# Autodesk Inventor assembly: Sneak100_Zeta
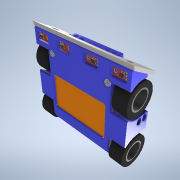
[picture p0: Inventor's stored thumbnail of the model, 180x180]
Saved by Autodesk Inventor 2021 (Build 250183000, 183)
## iProperties
Created: 2021-05-13
Part Number: Sneak100_Zeta
Document SubType Name: Assembly
Designer: ermoz
Author: ermoz
## Documents named in this file (15)
- D:\Moje Wyczyny\My_Poor_Projects\Sneak100_MiniSumo\minisumo-sneak100\mechanics\Sneak100_Zeta.iam
- D:\Moje Wyczyny\My_Poor_Projects\Sneak100_MiniSumo\minisumo-sneak100\mechanics\PreMadeParts\Pololu_MotorEncoderModule.iam
- D:\Moje Wyczyny\My_Poor_Projects\Sneak100_MiniSumo\minisumo-sneak100\mechanics\PreMadeParts\LiPO_2S_58x32x10.ipt
- D:\Moje Wyczyny\My_Poor_Projects\Sneak100_MiniSumo\minisumo-sneak100\mechanics\PreMadeParts\Solarbotics_RW2i.ipt
- D:\Moje Wyczyny\My_Poor_Projects\Sneak100_MiniSumo\minisumo-sneak100\mechanics\MechanicalElements\HullBottom.ipt
- D:\Moje Wyczyny\My_Poor_Projects\Sneak100_MiniSumo\minisumo-sneak100\mechanics\MechanicalElements\BatteryPlate.ipt
- D:\Moje Wyczyny\My_Poor_Projects\Sneak100_MiniSumo\minisumo-sneak100\mechanics\PreMadeParts\QTR1A.iam
- D:\Moje Wyczyny\My_Poor_Projects\Sneak100_MiniSumo\minisumo-sneak100\mechanics\PreMadeParts\M3_Short_Bolt.ipt
- D:\Moje Wyczyny\My_Poor_Projects\Sneak100_MiniSumo\minisumo-sneak100\mechanics\ModyfiedParts\HM_Knife_cut.ipt
- D:\Moje Wyczyny\My_Poor_Projects\Sneak100_MiniSumo\minisumo-sneak100\mechanics\PreMadeParts\3M_Nut.ipt
- D:\Moje Wyczyny\My_Poor_Projects\Sneak100_MiniSumo\minisumo-sneak100\mechanics\MechanicalElements\HullMid.ipt
- D:\Moje Wyczyny\My_Poor_Projects\Sneak100_MiniSumo\minisumo-sneak100\mechanics\MirroredParts\HullMid_MIR.ipt
- D:\Moje Wyczyny\My_Poor_Projects\Sneak100_MiniSumo\minisumo-sneak100\mechanics\MechanicalElements\HullTop.ipt
- D:\Moje Wyczyny\My_Poor_Projects\Sneak100_MiniSumo\minisumo-sneak100\mechanics\ElectricElements\MainModule.iam
- D:\Moje Wyczyny\My_Poor_Projects\Sneak100_MiniSumo\minisumo-sneak100\mechanics\PreMadeParts\M3_Long_Bolt.ipt
## Components (34 placed, 14 different names)
1. Pololu_MotorEncoderModule:1 [sub-assembly] — Mate:1, Flush:1, Flush:3, Flush:5, Angle:1, Mate:6, Mate:7, Symmetry:1
2. Pololu_MotorEncoderModule:2 [sub-assembly] — Mate:2, Flush:2, Flush:3, Flush:5, Angle:2, Mate:6, Mate:9, Mate:11, Mate:15, Mate:16
3. Pololu_MotorEncoderModule:3 [sub-assembly] — Mate:1, Flush:1, Flush:4, Mate:8, Symmetry:1
4. Pololu_MotorEncoderModule:4 [sub-assembly] — Mate:2, Flush:2, Flush:4, Mate:10, Mate:11
5. LiPO_2S_58x32x10:1 — Mate:17, Mate:18, Mate:70
6. Solarbotics_RW2i:1 — Mate:3, Tangent:1, Mate:7, Flush:8, Symmetry:2
7. Solarbotics_RW2i:2 — Tangent:2, Mate:9, Flush:8, Flush:11
8. Solarbotics_RW2i:3 — Mate:3, Mate:8, Flush:7, Symmetry:2, Flush:22
9. Solarbotics_RW2i:4 — Mate:10, Flush:7
10. HullBottom:1 — Flush:11, Mate:15, Mate:16, Mate:17, Mate:18, Mate:19, Mate:20, Mate:29, Flush:29, Flush:31, Mate:47, Mate:48, Flush:33, Mate:52, Mate:53, Mate:56, Mate:57, Mate:65, Mate:66, Mate:67, Mate:68, Mate:69, Mate:74, Mate:75, Flush:39
11. BatteryPlate:1 — Mate:19, Mate:20, Mate:69, Mate:70
12. QTR1A:1 [sub-assembly] — Symmetry:4, Flush:14, Flush:17, Mate:67, Mate:68
13. QTR1A:2 [sub-assembly] — Symmetry:3, Flush:13, Flush:14, Flush:16, Flush:17, Mate:65, Mate:66
14. QTR1A:3 [sub-assembly] — Symmetry:3, Flush:12, Flush:13, Flush:15, Flush:16
15. QTR1A:4 [sub-assembly] — Symmetry:4, Flush:12, Flush:15
16. M3_Short_Bolt:5 — Symmetry:5, Flush:23, Mate:31
17. M3_Short_Bolt:6 — Symmetry:5, Flush:24
18. HM_Knife_cut:1 — Mate:29, Flush:22, Flush:23, Mate:31, Flush:24
19. HullMid:1 — Mate:45, Mate:51, Mate:55, Flush:38, Mate:71, Mate:72, Mate:74, Mate:75, Mate:76
20. HullMid_MIR:1 — Flush:29, Mate:43, Mate:59, Flush:38, Mate:73
21. HullTop:1 — Flush:31, Mate:61, Mate:76, Flush:39
22. MainModule:1 [sub-assembly] — Mate:43, Mate:45, Mate:71, Mate:72, Mate:73
23. M3_Long_Bolt:1 — Mate:47, Flush:32, Flush:33, Mate:49, Mate:60
24. M3_Long_Bolt:2 — Mate:48, Flush:32, Mate:50, Mate:63
25. M3_Long_Bolt:3 — Mate:52, Mate:53, Mate:54, Mate:62
26. M3_Long_Bolt:4 — Mate:56, Mate:57, Mate:58, Mate:64
27. 3M_Nut:7 — Mate:49, Flush:34, Mate:51
28. 3M_Nut:8 — Mate:50, Flush:34
29. 3M_Nut:9 — Mate:54, Mate:55
30. 3M_Nut:10 — Mate:58, Mate:59
31. 3M_Nut:11 — Mate:60, Flush:35, Mate:61, Flush:37
32. 3M_Nut:12 — Mate:63, Flush:37
33. 3M_Nut:13 — Flush:35, Mate:62, Flush:36
34. 3M_Nut:14 — Flush:36, Mate:64
## Relationships (85: Mate 49, Flush 27, Symmetry 5, Angle 2, Tangent 2)
- Mate:1: Pololu_MotorEncoderModule:1 ↔ Pololu_MotorEncoderModule:3
- Flush:1: Pololu_MotorEncoderModule:1 ↔ Pololu_MotorEncoderModule:3
- Mate:2: Pololu_MotorEncoderModule:2 ↔ Pololu_MotorEncoderModule:4
- Flush:2: Pololu_MotorEncoderModule:2 ↔ Pololu_MotorEncoderModule:4
- Flush:3: Pololu_MotorEncoderModule:1 ↔ Pololu_MotorEncoderModule:2
- Flush:4: Pololu_MotorEncoderModule:3 ↔ Pololu_MotorEncoderModule:4
- Flush:5: Pololu_MotorEncoderModule:1 ↔ Pololu_MotorEncoderModule:2
- Mate:3 (-98 mm): Solarbotics_RW2i:1 ↔ Solarbotics_RW2i:3
- Angle:1 (0 deg): Pololu_MotorEncoderModule:1
- Tangent:1: Solarbotics_RW2i:1
- Angle:2 (0 deg): Pololu_MotorEncoderModule:2
- Tangent:2: Solarbotics_RW2i:2
- Mate:6 (50 mm): Pololu_MotorEncoderModule:1 ↔ Pololu_MotorEncoderModule:2
- Mate:7: Pololu_MotorEncoderModule:1 ↔ Solarbotics_RW2i:1
- Mate:8: Pololu_MotorEncoderModule:3 ↔ Solarbotics_RW2i:3
- Mate:9: Pololu_MotorEncoderModule:2 ↔ Solarbotics_RW2i:2
- Mate:10: Pololu_MotorEncoderModule:4 ↔ Solarbotics_RW2i:4
- Flush:7: Solarbotics_RW2i:3 ↔ Solarbotics_RW2i:4
- Flush:8: Solarbotics_RW2i:1 ↔ Solarbotics_RW2i:2
- Mate:11 (-68 mm): Pololu_MotorEncoderModule:2 ↔ Pololu_MotorEncoderModule:4
- Symmetry:1: Pololu_MotorEncoderModule:1 ↔ Pololu_MotorEncoderModule:3
- Symmetry:2: Solarbotics_RW2i:1 ↔ Solarbotics_RW2i:3
- Flush:11: Solarbotics_RW2i:2 ↔ HullBottom:1
- Mate:15: Pololu_MotorEncoderModule:2 ↔ HullBottom:1
- Mate:16: Pololu_MotorEncoderModule:2 ↔ HullBottom:1
- Mate:17: LiPO_2S_58x32x10:1 ↔ HullBottom:1
- Mate:18 (1 mm): LiPO_2S_58x32x10:1 ↔ HullBottom:1
- Mate:19: HullBottom:1 ↔ BatteryPlate:1
- Mate:20: HullBottom:1 ↔ BatteryPlate:1
- Symmetry:3: QTR1A:2 ↔ QTR1A:3
- Symmetry:4: QTR1A:1 ↔ QTR1A:4
- Flush:12: QTR1A:3 ↔ QTR1A:4
- Flush:13: QTR1A:2 ↔ QTR1A:3
- Flush:14: QTR1A:1 ↔ QTR1A:2
- Flush:15: QTR1A:3 ↔ QTR1A:4
- Flush:16: QTR1A:2 ↔ QTR1A:3
- Flush:17: QTR1A:1 ↔ QTR1A:2
- Symmetry:5: M3_Short_Bolt:5 ↔ M3_Short_Bolt:6
- Mate:29: HullBottom:1 ↔ HM_Knife_cut:1
- Flush:22 (-1 mm): Solarbotics_RW2i:3 ↔ HM_Knife_cut:1
- Flush:23: M3_Short_Bolt:5 ↔ HM_Knife_cut:1
- Mate:31: M3_Short_Bolt:5 ↔ HM_Knife_cut:1
- Flush:24: M3_Short_Bolt:6 ↔ HM_Knife_cut:1
- Flush:29: HullBottom:1 ↔ HullMid_MIR:1
- Mate:43: HullMid_MIR:1 ↔ MainModule:1
- Mate:45: HullMid:1 ↔ MainModule:1
- Flush:31: HullBottom:1 ↔ HullTop:1
- Mate:47: HullBottom:1 ↔ M3_Long_Bolt:1
- Mate:48: HullBottom:1 ↔ M3_Long_Bolt:2
- Flush:32: M3_Long_Bolt:1 ↔ M3_Long_Bolt:2
- Flush:33: HullBottom:1 ↔ M3_Long_Bolt:1
- Mate:49: M3_Long_Bolt:1 ↔ 3M_Nut:7
- Mate:50: M3_Long_Bolt:2 ↔ 3M_Nut:8
- Flush:34: 3M_Nut:7 ↔ 3M_Nut:8
- Mate:51: HullMid:1 ↔ 3M_Nut:7
- Mate:52: HullBottom:1 ↔ M3_Long_Bolt:3
- Mate:53: HullBottom:1 ↔ M3_Long_Bolt:3
- Mate:54: M3_Long_Bolt:3 ↔ 3M_Nut:9
- Mate:55: HullMid:1 ↔ 3M_Nut:9
- Mate:56: HullBottom:1 ↔ M3_Long_Bolt:4
- Mate:57: HullBottom:1 ↔ M3_Long_Bolt:4
- Mate:58: M3_Long_Bolt:4 ↔ 3M_Nut:10
- Mate:59: HullMid_MIR:1 ↔ 3M_Nut:10
- Mate:60: M3_Long_Bolt:1 ↔ 3M_Nut:11
- Flush:35: 3M_Nut:11 ↔ 3M_Nut:13
- Mate:61: HullTop:1 ↔ 3M_Nut:11
- Mate:62: M3_Long_Bolt:3 ↔ 3M_Nut:13
- Flush:36: 3M_Nut:13 ↔ 3M_Nut:14
- Mate:63: M3_Long_Bolt:2 ↔ 3M_Nut:12
- Flush:37: 3M_Nut:11 ↔ 3M_Nut:12
- Mate:64: M3_Long_Bolt:4 ↔ 3M_Nut:14
- Mate:65: HullBottom:1 ↔ QTR1A:2
- Mate:66: HullBottom:1 ↔ QTR1A:2
- Mate:67: HullBottom:1 ↔ QTR1A:1
- Mate:68: HullBottom:1 ↔ QTR1A:1
- Mate:69: HullBottom:1 ↔ BatteryPlate:1
- Mate:70: LiPO_2S_58x32x10:1 ↔ BatteryPlate:1
- Flush:38: HullMid:1 ↔ HullMid_MIR:1
- Mate:71: HullMid:1 ↔ MainModule:1
- Mate:72: HullMid:1 ↔ MainModule:1
- Mate:73: HullMid_MIR:1 ↔ MainModule:1
- Mate:74: HullBottom:1 ↔ HullMid:1
- Mate:75: HullBottom:1 ↔ HullMid:1
- Mate:76: HullMid:1 ↔ HullTop:1
- Flush:39: HullBottom:1 ↔ HullTop:1
